# Autodesk Inventor assembly: Intake
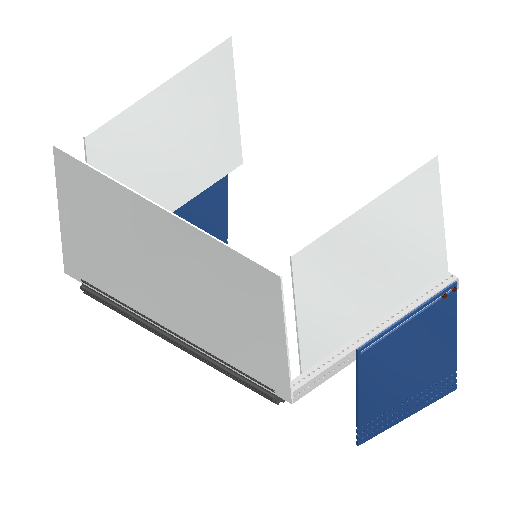
[picture p0: Inventor's stored thumbnail of the model, 512x512]
Saved by Autodesk Inventor 2025.3 (Build 293356000, 356)
## iProperties
Created: 2026-05-13
Part Number: Intake
Document SubType Name: Assembly
Designer: djair.oliveira
Author: djair.oliveira
## Documents named in this file (8)
- C:\Users\djair.oliveira\Documents\GitHub\MT_2026\CAD\Model A\Intake\Intake.iam
- C:\Users\djair.oliveira\Documents\GitHub\MT_2026\CAD\Model A\Intake\Guia - Intake.ipt
- C:\Users\djair.oliveira\Documents\GitHub\MT_2026\CAD\Model A\Intake\Move - Intake.ipt
- C:\Users\djair.oliveira\Documents\GitHub\MT_2026\CAD\Model A\Intake\Coletor - Intake.ipt
- C:\Users\djair.oliveira\Documents\GitHub\MT_2026\CAD\Model A\Intake\Chapa Frontal - Intake.ipt
- C:\Users\djair.oliveira\Documents\GitHub\MT_2026\CAD\Model A\Intake\Chapa Lateral - Intake.ipt
- C:\Users\djair.oliveira\Documents\GitHub\MT_2026\CAD\Model A\Intake\Suporte Guia - Intake.ipt
- C:\Users\djair.oliveira\Documents\GitHub\MT_2026\CAD\Model A\Intake\Suporte Coletor - Intake.ipt
## Components (14 placed, 7 different names)
1. Guia - Intake:1 — Coincidente:1, Coincidente:2, Coincidente:3, Coincidente:4, Tangente:1, Tangente:2
2. Guia - Intake:2 — Coincidente:1, Coincidente:2, Coincidente:3, Coincidente:13, Coincidente:18
3. Move - Intake:1 — Coincidente:4, Tangente:1, Tangente:2, Alinhado:1, Alinhado:2, Coincidente:22, Coincidente:23, Coincidente:24, Coincidente:27, Alinhado:3, Alinhado:4, Alinhado:5, Coincidente:28, Alinhado:6, Coincidente:30, Coincidente:31, Coincidente:32, Coincidente:33
4. Move - Intake:2 — Coincidente:13, Alinhado:1, Alinhado:2, Coincidente:18, Coincidente:19, Coincidente:20, Coincidente:21, Coincidente:29, Alinhado:7, Alinhado:8, Coincidente:34, Coincidente:35, Coincidente:36, Coincidente:37
5. Coletor - Intake:1 — Coincidente:25, Coincidente:26
6. Chapa Frontal - Intake:1 — Coincidente:27, Alinhado:3, Alinhado:4
7. Chapa Lateral - Intake:1 — Coincidente:29, Alinhado:7, Alinhado:8
8. Chapa Lateral - Intake:2 — Alinhado:5, Coincidente:28, Alinhado:6
9. Suporte Coletor - Intake:1 — Coincidente:22, Coincidente:23, Coincidente:24, Coincidente:25
10. Suporte Coletor - Intake:2 — Coincidente:19, Coincidente:20, Coincidente:21, Coincidente:26
11. Suporte Guia - Intake:1 — Coincidente:34, Coincidente:36
12. Suporte Guia - Intake:2 — Coincidente:35, Coincidente:37
13. Suporte Guia - Intake:3 — Coincidente:31, Coincidente:32
14. Suporte Guia - Intake:4 — Coincidente:30, Coincidente:33
## Relationships (35: Mate 25, Flush 8, Tangent 2)
- Coincidente:1 [Mate] (584.2 mm): Guia - Intake:1 ↔ Guia - Intake:2
- Coincidente:2 [Mate]: Guia - Intake:1 ↔ Guia - Intake:2
- Coincidente:3 [Mate]: Guia - Intake:1 ↔ Guia - Intake:2
- Coincidente:4 [Mate]: Guia - Intake:1 ↔ Move - Intake:1
- Tangente:1 (0.5 mm): Guia - Intake:1 ↔ Move - Intake:1
- Tangente:2 (0.5 mm): Guia - Intake:1 ↔ Move - Intake:1
- Coincidente:13 [Mate]: Guia - Intake:2 ↔ Move - Intake:2
- Alinhado:1 [Flush]: Move - Intake:1 ↔ Move - Intake:2
- Alinhado:2 [Flush]: Move - Intake:1 ↔ Move - Intake:2
- Coincidente:18 [Mate]: Guia - Intake:2 ↔ Move - Intake:2
- Coincidente:19 [Mate]: Move - Intake:2 ↔ Suporte Coletor - Intake:2
- Coincidente:20 [Mate]: Move - Intake:2 ↔ Suporte Coletor - Intake:2
- Coincidente:21 [Mate]: Move - Intake:2 ↔ Suporte Coletor - Intake:2
- Coincidente:22 [Mate]: Move - Intake:1 ↔ Suporte Coletor - Intake:1
- Coincidente:23 [Mate]: Move - Intake:1 ↔ Suporte Coletor - Intake:1
- Coincidente:24 [Mate]: Move - Intake:1 ↔ Suporte Coletor - Intake:1
- Coincidente:25 [Mate]: Coletor - Intake:1 ↔ Suporte Coletor - Intake:1
- Coincidente:26 [Mate]: Coletor - Intake:1 ↔ Suporte Coletor - Intake:2
- Coincidente:27 [Mate]: Move - Intake:1 ↔ Chapa Frontal - Intake:1
- Alinhado:3 [Flush]: Move - Intake:1 ↔ Chapa Frontal - Intake:1
- Alinhado:4 [Flush]: Move - Intake:1 ↔ Chapa Frontal - Intake:1
- Alinhado:5 [Flush]: Move - Intake:1 ↔ Chapa Lateral - Intake:2
- Coincidente:28 [Mate]: Move - Intake:1 ↔ Chapa Lateral - Intake:2
- Alinhado:6 [Flush]: Move - Intake:1 ↔ Chapa Lateral - Intake:2
- Coincidente:29 [Mate]: Move - Intake:2 ↔ Chapa Lateral - Intake:1
- Alinhado:7 [Flush]: Move - Intake:2 ↔ Chapa Lateral - Intake:1
- Alinhado:8 [Flush]: Move - Intake:2 ↔ Chapa Lateral - Intake:1
- Coincidente:30 [Mate]: Move - Intake:1 ↔ Suporte Guia - Intake:4
- Coincidente:31 [Mate]: Move - Intake:1 ↔ Suporte Guia - Intake:3
- Coincidente:32 [Mate]: Move - Intake:1 ↔ Suporte Guia - Intake:3
- Coincidente:33 [Mate]: Move - Intake:1 ↔ Suporte Guia - Intake:4
- Coincidente:34 [Mate]: Move - Intake:2 ↔ Suporte Guia - Intake:1
- Coincidente:35 [Mate]: Move - Intake:2 ↔ Suporte Guia - Intake:2
- Coincidente:36 [Mate]: Move - Intake:2 ↔ Suporte Guia - Intake:1
- Coincidente:37 [Mate]: Move - Intake:2 ↔ Suporte Guia - Intake:2
